# Autodesk Inventor assembly: Conjunto transimisión
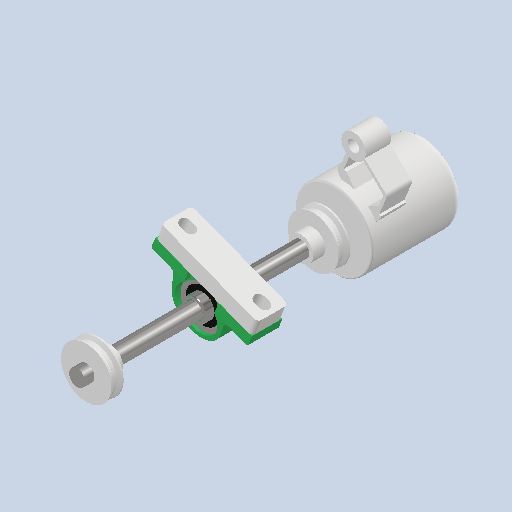
[picture p0: Inventor's stored thumbnail of the model, 512x512]
Saved by Autodesk Inventor 2022 (Build 260153000, 153)
## iProperties
Created: 2019-10-25
Part Number: Conjunto transimisión
Document SubType Name: Assembly
Designer: Usuario
Author: Usuario
## Documents named in this file (7)
- G:\Mi unidad\UTEC\Proyectos\Flor de Lana\Diseño 20191119\Conjunto transimisión.iam
- G:\Mi unidad\UTEC\Proyectos\Flor de Lana\Diseño 20191119\UCP-204.ipt
- G:\Mi unidad\UTEC\Proyectos\Flor de Lana\Diseño 20191119\Eje_Base.ipt
- G:\Mi unidad\UTEC\Proyectos\Flor de Lana\Diseño 20191119\SoporteMancal.ipt
- G:\Mi unidad\UTEC\Proyectos\Flor de Lana\Diseño 20191119\PoleaBrazos.ipt
- G:\Mi unidad\UTEC\Proyectos\Flor de Lana\Diseño 20191119\motor.ipt
- G:\Mi unidad\UTEC\Proyectos\Flor de Lana\Diseño 20191119\PoleaMotor.ipt
## Components (6 placed, 6 different names)
1. UCP-204:1 — Cilíndrica:2, Rígido:1
2. Eje_Base:1 — Cilíndrica:2, De rotación:3, De rotación:4, Rigid:2
3. SoporteMancal:1 — Rígido:1
4. PoleaBrazos:1 — De rotación:3
5. motor:1 — De rotación:4
6. PoleaMotor:1 — Rigid:2
## Relationships (5: WeldJoint 2, RevoluteJoint 2, CylindricalJoint 1)
- Cilíndrica:2 [CylindricalJoint]: UCP-204:1 ↔ Eje_Base:1
- Rígido:1 [WeldJoint] (1.5 mm): UCP-204:1 ↔ SoporteMancal:1
- De rotación:3 [RevoluteJoint] (-41 mm): Eje_Base:1 ↔ PoleaBrazos:1
- De rotación:4 [RevoluteJoint]: Eje_Base:1 ↔ motor:1
- Rigid:2 [WeldJoint] (-15 mm): Eje_Base:1 ↔ PoleaMotor:1
